# Autodesk Inventor assembly: Shooter Mount6000
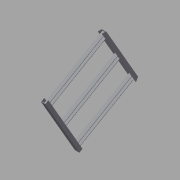
[picture p0: Inventor's stored thumbnail of the model, 180x180]
Saved by Autodesk Inventor 2013 (Build 170138000, 138)
## iProperties
Created: 2013-01-09
Part Number: Shooter Mount6000
Document SubType Name: Assembly
Designer: Naphat
Author: Naphat
## Documents named in this file (3)
- C:\Autodesk\Shooter Mount6000-cad\Shooter Mount6000.iam
- C:\Autodesk\Shooter Mount6000-cad\19in c-channel.ipt
- C:\Autodesk\Shooter Mount6000-cad\19in c-channel-top.ipt
## Components (5 placed, 2 different names)
1. 19in c-channel:1 — Mate:25, Mate:26, Flush:4
2. 19in c-channel:2 — Mate:23, Mate:24, Flush:5
3. 19in c-channel:3 — Mate:21, Mate:22, Mate:23, Mate:24, Mate:25, Mate:26, Flush:3, Flush:4, Flush:5
4. 19in c-channel:5 — Mate:21, Mate:22, Flush:3, Mate:27, Mate:28
5. 19in c-channel-top:1 — Mate:27, Mate:28
## Relationships (11: Mate 8, Flush 3)
- Mate:21: 19in c-channel:3 ↔ 19in c-channel:5
- Mate:22: 19in c-channel:3 ↔ 19in c-channel:5
- Mate:23: 19in c-channel:2 ↔ 19in c-channel:3
- Mate:24: 19in c-channel:2 ↔ 19in c-channel:3
- Mate:25: 19in c-channel:1 ↔ 19in c-channel:3
- Mate:26: 19in c-channel:1 ↔ 19in c-channel:3
- Flush:3 (25.4 mm): 19in c-channel:3 ↔ 19in c-channel:5
- Flush:4 (25.4 mm): 19in c-channel:1 ↔ 19in c-channel:3
- Flush:5 (225.6 mm): 19in c-channel:2 ↔ 19in c-channel:3
- Mate:27: 19in c-channel:5 ↔ 19in c-channel-top:1
- Mate:28: 19in c-channel:5 ↔ 19in c-channel-top:1
